# Autodesk Inventor assembly: Fullsystem_V015
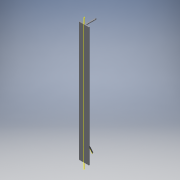
[picture p0: Inventor's stored thumbnail of the model, 180x180]
Saved by Autodesk Inventor 2016 (Build 200138000, 138)
## iProperties
Created: 2016-11-07
Part Number: Fullsystem_V015
Document SubType Name: Assembly
Designer: Matt Cocca
Author: Matt Cocca
## Documents named in this file (4)
- C:\Users\mattc\OneDrive\Documents\Inventor\EmbeddedBalance\Fullsystem_V015.iam
- C:\Users\mattc\OneDrive\Documents\Inventor\EmbeddedBalance\Base_015.ipt
- C:\Users\mattc\OneDrive\Documents\Inventor\EmbeddedBalance\Servo.ipt
- C:\Users\mattc\OneDrive\Documents\Inventor\EmbeddedBalance\ServoLinkage_015.ipt
## Components (3 placed, 3 different names)
1. Base_015:1 — Mate:1, Mate:2, Mate:3
2. Servo:1 — Mate:1, Mate:2, Mate:3, Insert:1
3. ServoLinkage_015:1 — Insert:1
## Relationships (4: Mate 3, Insert 1)
- Mate:1: Base_015:1 ↔ Servo:1
- Mate:2: Base_015:1 ↔ Servo:1
- Mate:3: Base_015:1 ↔ Servo:1
- Insert:1 (1 mm): Servo:1 ↔ ServoLinkage_015:1
